# Autodesk Inventor assembly: Mao-robotica-alpha-costas
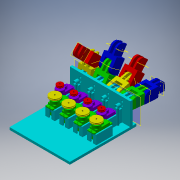
[picture p0: Inventor's stored thumbnail of the model, 180x180]
Saved by Autodesk Inventor 2018 (Build 220112000, 112)
## iProperties
Created: 2017-06-05
Part Number: Mao-robotica-alpha-costas
Material: Genérico
Document SubType Name: Assembly
Designer: Vitor
Author: Vitor
## Documents named in this file (6)
- C:\Users\Vitor\Documents\Autodesk\Mao-Robotica\Mao-robotica-alpha-costas.iam
- C:\Users\Vitor\Documents\Autodesk\Mao-Robotica\Costas.ipt
- C:\Users\Vitor\Documents\Autodesk\Mao-Robotica\Motor.ipt
- C:\Users\Vitor\Documents\Autodesk\Mao-Robotica\Polia.ipt
- C:\Users\Vitor\Documents\Autodesk\Mao-Robotica\Polia2.ipt
- C:\Users\Vitor\Documents\Autodesk\Mao-Robotica\Falange-media2.ipt
## Components (25 placed, 5 different names)
1. Costas:1 — Inserir:1, Inserir:2, Inserir:3, Inserir:4, Inserir:5, Inserir:6, Inserir:7, Inserir:8, Inserir:9, Inserir:10, Inserir:11, Inserir:12, Inserir:13, Inserir:14, Inserir:15, Inserir:16, Inserir:26, Inserir:27, Inserir:28, Inserir:29
2. Motor:1 — Inserir:9, Inserir:10, Inserir:19
3. Motor:2 — Inserir:7, Inserir:8, Inserir:22
4. Motor:3 — Inserir:1, Inserir:2, Inserir:17
5. Motor:4 — Inserir:3, Inserir:4, Inserir:21
6. Motor:5 — Inserir:15, Inserir:16, Inserir:24
7. Motor:6 — Inserir:13, Inserir:14, Inserir:20
8. Motor:7 — Inserir:11, Inserir:12, Inserir:23
9. Motor:8 — Inserir:5, Inserir:6, Inserir:18
10. Polia:1 — Inserir:17
11. Polia:2 — Inserir:18
12. Polia:3 — Inserir:19
13. Polia:4 — Inserir:20
14. Polia2:1 — Inserir:23
15. Polia2:2 — Inserir:22
16. Polia2:3 — Inserir:24
17. Polia2:4 — Inserir:21
18. Falange-media2:1 — Inserir:25
19. Falange-media2:2 — Inserir:25, Inserir:26
20. Falange-media2:3 — Inserir:27, Inserir:31
21. Falange-media2:4 — Inserir:29, Inserir:32
22. Falange-media2:5 — Inserir:32
23. Falange-media2:6 — Inserir:31
24. Falange-media2:7 — Inserir:28, Inserir:30
25. Falange-media2:8 — Inserir:30
## Relationships (32: Insert 32)
- Inserir:1: Costas:1 ↔ Motor:3
- Inserir:2: Costas:1 ↔ Motor:3
- Inserir:3: Costas:1 ↔ Motor:4
- Inserir:4: Costas:1 ↔ Motor:4
- Inserir:5: Costas:1 ↔ Motor:8
- Inserir:6: Costas:1 ↔ Motor:8
- Inserir:7: Costas:1 ↔ Motor:2
- Inserir:8: Costas:1 ↔ Motor:2
- Inserir:9: Costas:1 ↔ Motor:1
- Inserir:10: Costas:1 ↔ Motor:1
- Inserir:11: Costas:1 ↔ Motor:7
- Inserir:12: Costas:1 ↔ Motor:7
- Inserir:13: Costas:1 ↔ Motor:6
- Inserir:14: Costas:1 ↔ Motor:6
- Inserir:15: Costas:1 ↔ Motor:5
- Inserir:16: Costas:1 ↔ Motor:5
- Inserir:17: Motor:3 ↔ Polia:1
- Inserir:18: Motor:8 ↔ Polia:2
- Inserir:19: Motor:1 ↔ Polia:3
- Inserir:20: Motor:6 ↔ Polia:4
- Inserir:21: Motor:4 ↔ Polia2:4
- Inserir:22: Motor:2 ↔ Polia2:2
- Inserir:23: Motor:7 ↔ Polia2:1
- Inserir:24: Motor:5 ↔ Polia2:3
- Inserir:25 (0.5 mm): Falange-media2:1 ↔ Falange-media2:2
- Inserir:26 (0.5 mm): Costas:1 ↔ Falange-media2:2
- Inserir:27 (0.5 mm): Costas:1 ↔ Falange-media2:3
- Inserir:28 (0.5 mm): Costas:1 ↔ Falange-media2:7
- Inserir:29 (0.5 mm): Costas:1 ↔ Falange-media2:4
- Inserir:30 (0.5 mm): Falange-media2:7 ↔ Falange-media2:8
- Inserir:31 (0.5 mm): Falange-media2:3 ↔ Falange-media2:6
- Inserir:32 (0.5 mm): Falange-media2:4 ↔ Falange-media2:5
